# Autodesk Inventor assembly: enc-TopPanel V2 - Assembly no Absorber
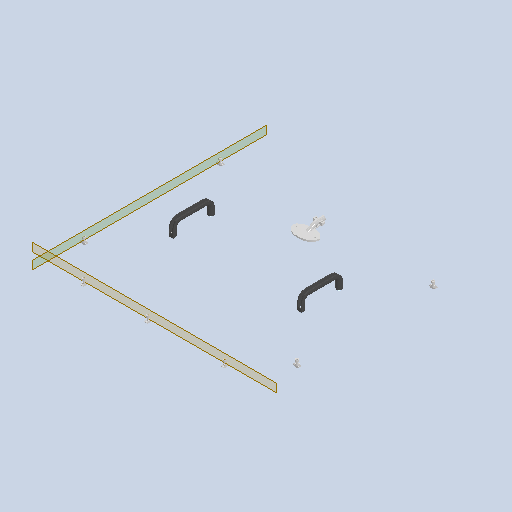
[picture p0: Inventor's stored thumbnail of the model, 512x512]
Saved by Autodesk Inventor 2023.2 (Build 272271000, 271)
## iProperties
Created: 2023-12-13
Part Number: enc-TopPanel V2 - Assembly no Absorber
Document SubType Name: Assembly
Designer: Nils Bade
Author: Nils Bade
## Documents named in this file (5)
- C:\Users\nilsb\Documents\Inventor\Projektarbeit-Bade\Enclosure\enc-TopPanel V2 - Assembly no Absorber.iam
- C:\Users\nilsb\Documents\Inventor\Projektarbeit-Bade\Enclosure\enc-TopPanel V2.ipt
- C:\Users\nilsb\Documents\Inventor\Projektarbeit-Bade\Schrauben\Cap Head Screw M6x12 v2.ipt
- C:\Users\nilsb\Documents\Inventor\Projektarbeit-Bade\RatRig_modified\T-NUT - DropIn 4040 SERIES - M6.ipt
- C:\Users\nilsb\Documents\Inventor\Projektarbeit-Bade\Enclosure\item_Handgriff_PA120_Assembly.iam
## Components (17 placed, 4 different names)
1. enc-TopPanel V2 - 710x678:1 — Einfügen:1, Einfügen:2, Einfügen:3, Einfügen:4, Einfügen:5, Einfügen:6, Einfügen:7, Passend:22, Passend:23, Passend:24, Passend:25, Passend:26, Passend:27, Passend:28, Winkel:1, Winkel:2, Winkel:3, Winkel:4, Winkel:5, Winkel:6, Winkel:7, Passend:35, Passend:36, Passend:37, Passend:38, Passend:39, Passend:40, Fluchtend:1, Fluchtend:2
2. Cap Head Screw M6x12 v2:1 — Einfügen:2, Passend:20
3. Cap Head Screw M6x12 v2:2 — Einfügen:3, Passend:19
4. Cap Head Screw M6x12 v2:3 — Einfügen:1, Passend:21
5. Cap Head Screw M6x12 v2:4 — Einfügen:4, Passend:18
6. Cap Head Screw M6x12 v2:5 — Einfügen:7, Passend:17
7. Cap Head Screw M6x12 v2:6 — Einfügen:6, Passend:16
8. Cap Head Screw M6x12 v2:7 — Einfügen:5, Passend:15
9. T-NUT - DROP IN TYPE FOR 40 SERIES - M6:1 — Passend:18, Passend:27, Winkel:2
10. T-NUT - DROP IN TYPE FOR 40 SERIES - M6:2 — Passend:19, Passend:28, Winkel:1
11. T-NUT - DROP IN TYPE FOR 40 SERIES - M6:3 — Passend:21, Passend:22, Winkel:6
12. T-NUT - DROP IN TYPE FOR 40 SERIES - M6:4 — Passend:20, Passend:23, Winkel:7
13. T-NUT - DROP IN TYPE FOR 40 SERIES - M6:5 — Passend:17, Passend:24, Winkel:5
14. T-NUT - DROP IN TYPE FOR 40 SERIES - M6:6 — Passend:16, Passend:25, Winkel:4
15. T-NUT - DROP IN TYPE FOR 40 SERIES - M6:7 — Passend:15, Passend:26, Winkel:3
16. item_Handgriff_120er:1 [sub-assembly] — Passend:35, Passend:36, Passend:39
17. item_Handgriff_120er:2 [sub-assembly] — Passend:37, Passend:38, Passend:40
## Relationships (36: Mate 20, Insert 7, Angle 7, Flush 2)
- Einfügen:1 [Insert]: enc-TopPanel V2 - 710x678:1 ↔ Cap Head Screw M6x12 v2:3
- Einfügen:2 [Insert]: enc-TopPanel V2 - 710x678:1 ↔ Cap Head Screw M6x12 v2:1
- Einfügen:3 [Insert]: enc-TopPanel V2 - 710x678:1 ↔ Cap Head Screw M6x12 v2:2
- Einfügen:4 [Insert]: enc-TopPanel V2 - 710x678:1 ↔ Cap Head Screw M6x12 v2:4
- Einfügen:5 [Insert]: enc-TopPanel V2 - 710x678:1 ↔ Cap Head Screw M6x12 v2:7
- Einfügen:6 [Insert]: enc-TopPanel V2 - 710x678:1 ↔ Cap Head Screw M6x12 v2:6
- Einfügen:7 [Insert]: enc-TopPanel V2 - 710x678:1 ↔ Cap Head Screw M6x12 v2:5
- Passend:15 [Mate]: Cap Head Screw M6x12 v2:7 ↔ T-NUT - DROP IN TYPE FOR 40 SERIES - M6:7
- Passend:16 [Mate]: Cap Head Screw M6x12 v2:6 ↔ T-NUT - DROP IN TYPE FOR 40 SERIES - M6:6
- Passend:17 [Mate]: Cap Head Screw M6x12 v2:5 ↔ T-NUT - DROP IN TYPE FOR 40 SERIES - M6:5
- Passend:18 [Mate]: Cap Head Screw M6x12 v2:4 ↔ T-NUT - DROP IN TYPE FOR 40 SERIES - M6:1
- Passend:19 [Mate]: Cap Head Screw M6x12 v2:2 ↔ T-NUT - DROP IN TYPE FOR 40 SERIES - M6:2
- Passend:20 [Mate]: Cap Head Screw M6x12 v2:1 ↔ T-NUT - DROP IN TYPE FOR 40 SERIES - M6:4
- Passend:21 [Mate]: Cap Head Screw M6x12 v2:3 ↔ T-NUT - DROP IN TYPE FOR 40 SERIES - M6:3
- Passend:22 [Mate] (5.5 mm): enc-TopPanel V2 - 710x678:1 ↔ T-NUT - DROP IN TYPE FOR 40 SERIES - M6:3
- Passend:23 [Mate] (5.5 mm): enc-TopPanel V2 - 710x678:1 ↔ T-NUT - DROP IN TYPE FOR 40 SERIES - M6:4
- Passend:24 [Mate] (5.5 mm): enc-TopPanel V2 - 710x678:1 ↔ T-NUT - DROP IN TYPE FOR 40 SERIES - M6:5
- Passend:25 [Mate] (5.5 mm): enc-TopPanel V2 - 710x678:1 ↔ T-NUT - DROP IN TYPE FOR 40 SERIES - M6:6
- Passend:26 [Mate] (5.5 mm): enc-TopPanel V2 - 710x678:1 ↔ T-NUT - DROP IN TYPE FOR 40 SERIES - M6:7
- Passend:27 [Mate] (5.5 mm): enc-TopPanel V2 - 710x678:1 ↔ T-NUT - DROP IN TYPE FOR 40 SERIES - M6:1
- Passend:28 [Mate] (5.5 mm): enc-TopPanel V2 - 710x678:1 ↔ T-NUT - DROP IN TYPE FOR 40 SERIES - M6:2
- Winkel:1 [Angle] (0 deg): enc-TopPanel V2 - 710x678:1 ↔ T-NUT - DROP IN TYPE FOR 40 SERIES - M6:2
- Winkel:2 [Angle] (0 deg): enc-TopPanel V2 - 710x678:1 ↔ T-NUT - DROP IN TYPE FOR 40 SERIES - M6:1
- Winkel:3 [Angle] (0 deg): enc-TopPanel V2 - 710x678:1 ↔ T-NUT - DROP IN TYPE FOR 40 SERIES - M6:7
- Winkel:4 [Angle] (0 deg): enc-TopPanel V2 - 710x678:1 ↔ T-NUT - DROP IN TYPE FOR 40 SERIES - M6:6
- Winkel:5 [Angle] (0 deg): enc-TopPanel V2 - 710x678:1 ↔ T-NUT - DROP IN TYPE FOR 40 SERIES - M6:5
- Winkel:6 [Angle] (0 deg): enc-TopPanel V2 - 710x678:1 ↔ T-NUT - DROP IN TYPE FOR 40 SERIES - M6:3
- Winkel:7 [Angle] (0 deg): enc-TopPanel V2 - 710x678:1 ↔ T-NUT - DROP IN TYPE FOR 40 SERIES - M6:4
- Passend:35 [Mate]: enc-TopPanel V2 - 710x678:1 ↔ item_Handgriff_120er:1
- Passend:36 [Mate]: enc-TopPanel V2 - 710x678:1 ↔ item_Handgriff_120er:1
- Passend:37 [Mate]: enc-TopPanel V2 - 710x678:1 ↔ item_Handgriff_120er:2
- Passend:38 [Mate]: enc-TopPanel V2 - 710x678:1 ↔ item_Handgriff_120er:2
- Passend:39 [Mate]: enc-TopPanel V2 - 710x678:1 ↔ item_Handgriff_120er:1
- Passend:40 [Mate]: enc-TopPanel V2 - 710x678:1 ↔ item_Handgriff_120er:2
- Fluchtend:1 [Flush] (-15 mm): enc-TopPanel V2 - 710x678:1
- Fluchtend:2 [Flush] (-15 mm): enc-TopPanel V2 - 710x678:1
